# Autodesk Inventor assembly: Assembly1
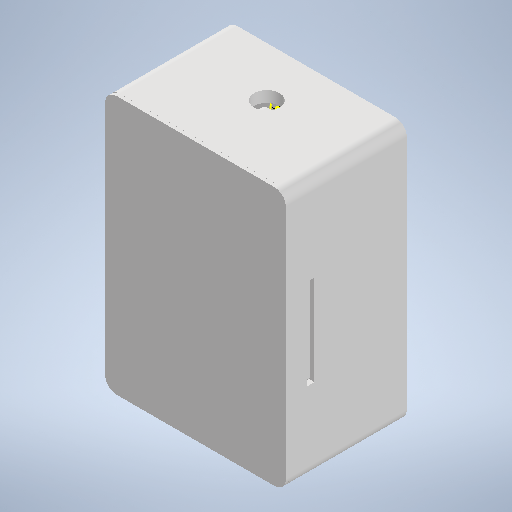
[picture p0: Inventor's stored thumbnail of the model, 512x512]
Saved by Autodesk Inventor 2025.2 (Build 292293000, 293)
## iProperties
Created: 2022-04-10
Part Number: Assembly1
Document SubType Name: Assembly
Designer: Frizz
Author: Frizz
## Documents named in this file (4)
- C:\Users\Fred\OneDrive - University of California, Davis\Development\TracerGas Lite\3D Printed case\Assembly1.iam
- C:\Users\Fred\OneDrive - University of California, Davis\Development\TracerGas Lite\3D Printed case\CaseV2.ipt
- C:\Users\Fred\OneDrive - University of California, Davis\Development\TracerGas Lite\3D Printed case\Adafruit FONA Feather 32u4 v1.ipt
- C:\Users\Fred\OneDrive - University of California, Davis\Development\TracerGas Lite\3D Printed case\lidV2.ipt
## Components (3 placed, 3 different names)
1. caseV2 — Flush:1, Flush:2, Flush:3, Mate:1, Mate:2, Mate:3, Angle:1, Flush:4, Flush:5
2. Adafruit FONA Feather 32u4 v1:1 — Mate:1, Mate:2, Mate:4
3. lidV2:1 — Flush:4, Flush:5
## Relationships (10: Flush 5, Mate 4, Angle 1)
- Flush:1: caseV2
- Flush:2: caseV2
- Flush:3: caseV2
- Mate:1: caseV2 ↔ Adafruit FONA Feather 32u4 v1:1
- Mate:2 (3.175 mm): caseV2 ↔ Adafruit FONA Feather 32u4 v1:1
- Mate:3: caseV2
- Angle:1 (0 deg): caseV2
- Mate:4: Adafruit FONA Feather 32u4 v1:1
- Flush:4: caseV2 ↔ lidV2:1
- Flush:5: caseV2 ↔ lidV2:1
